# Autodesk Inventor assembly: s-assy-pillar2
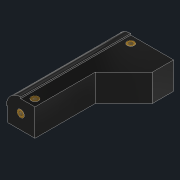
[picture p0: Inventor's stored thumbnail of the model, 180x180]
Saved by Autodesk Inventor 2021 (Build 250183000, 183)
## iProperties
Created: 2021-08-04
Part Number: s-assy-pillar2
Document SubType Name: Assembly
Designer: yuta0
Author: yuta0
## Documents named in this file (4)
- C:\Users\yuta0\Documents\GitHub\catchrobo_hardware\assy-robot\s-assy-pillar2.iam
- C:\Users\yuta0\Documents\GitHub\catchrobo_hardware\assy-robot\base5.ipt
- C:\Users\yuta0\Documents\GitHub\catchrobo_hardware\assy-robot\SB-305060.ipt
- C:\Users\yuta0\Documents\GitHub\catchrobo_hardware\assy-robot\holder_magnet.ipt
## Components (8 placed, 3 different names)
1. base5:1 — メイト:1, メイト:3, メイト:4, メイト:6, メイト:12, メイト:13, フラッシュ:1, フラッシュ:2, フラッシュ:3, フラッシュ:4
2. SB-305060:3 — メイト:3, フラッシュ:4
3. SB-305060:4 — メイト:4, フラッシュ:1
4. holder_magnet:1 — メイト:12, メイト:13
5. SB-305060:5 — メイト:6, フラッシュ:2
6. SB-305060:1 — メイト:1, フラッシュ:3
7. SB-305060:6
8. SB-305060:7
## Component patterns: (2 elements, first: SB-305060:5 + SB-305060:1)
## Relationships (10: Mate 6, Flush 4)
- メイト:1 [Mate]: base5:1 ↔ SB-305060:1
- メイト:3 [Mate]: base5:1 ↔ SB-305060:3
- メイト:4 [Mate]: base5:1 ↔ SB-305060:4
- メイト:6 [Mate]: base5:1 ↔ SB-305060:5
- メイト:12 [Mate]: base5:1 ↔ holder_magnet:1
- メイト:13 [Mate]: base5:1 ↔ holder_magnet:1
- フラッシュ:1 [Flush]: base5:1 ↔ SB-305060:4
- フラッシュ:2 [Flush]: base5:1 ↔ SB-305060:5
- フラッシュ:3 [Flush]: base5:1 ↔ SB-305060:1
- フラッシュ:4 [Flush]: base5:1 ↔ SB-305060:3
